# Autodesk Inventor assembly: Final assembly cuz we cool
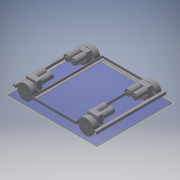
[picture p0: Inventor's stored thumbnail of the model, 180x180]
Saved by Autodesk Inventor 2016 SP2 (Build 200236200, 236)
## iProperties
Created: 2018-01-20
Part Number: Final assembly cuz we cool
Document SubType Name: Assembly
Designer: CAD
Author: CAD
## Documents named in this file (6)
- C:\Users\CAD\Documents\GitHub\FIRST-ROBOTICS-2018-5436-CAD\Robot\Chassis\Final assembly cuz we cool.iam
- C:\Users\CAD\Documents\GitHub\FIRST-ROBOTICS-2018-5436-CAD\Robot\Chassis\27.5 L.ipt
- C:\Users\CAD\Documents\GitHub\FIRST-ROBOTICS-2018-5436-CAD\Robot\Chassis\17.25 L.ipt
- C:\Users\CAD\Documents\GitHub\FIRST-ROBOTICS-2018-5436-CAD\Robot\Chassis\transmission with brackets.iam
- C:\Users\CAD\Documents\GitHub\FIRST-ROBOTICS-2018-5436-CAD\Robot\Chassis\Temp Wheels.ipt
- C:\Users\CAD\Documents\GitHub\FIRST-ROBOTICS-2018-5436-CAD\Robot\Chassis\27 in sq frame.ipt
## Components (14 placed, 5 different names)
1. 27.5 L:1 — Mate:9, Mate:10, Mate:25, Mate:26, Mate:29, Mate:30, Flush:2, Flush:3, Mate:32, Flush:4, Flush:5
2. transmission with brackets:1 [sub-assembly] — Mate:11, Mate:18, Mate:19, Mate:23
3. transmission with brackets:2 [sub-assembly] — Mate:10, Mate:12, Mate:17, Mate:20, Mate:24
4. transmission with brackets:3 [sub-assembly] — Mate:14, Mate:15, Mate:21
5. transmission with brackets:4 [sub-assembly] — Mate:9, Mate:13, Mate:16, Mate:22
6. Temp Wheels:1 — Mate:11, Mate:18, Mate:19
7. Temp Wheels:2 — Mate:13, Mate:16, Mate:22, Tangent:2
8. Temp Wheels:3 — Mate:14, Mate:15, Mate:21
9. Temp Wheels:4 — Mate:12, Mate:17, Mate:20
10. 27 in sq frame:1 — Mate:24
11. 27 in sq frame:2 — Mate:23, Angle:2
12. 17.25 L:1 — Mate:29, Mate:30, Flush:2, Mate:31, Flush:5, Mate:33, Flush:6
13. 17.25 L:2 — Mate:25, Mate:26, Flush:3, Mate:32, Flush:4
14. 27.5 L:2 — Mate:31, Mate:33, Flush:6
## Relationships (30: Mate 23, Flush 5, Angle 1, Tangent 1)
- Mate:9: 27.5 L:1 ↔ transmission with brackets:4
- Mate:10: 27.5 L:1 ↔ transmission with brackets:2
- Mate:11: transmission with brackets:1 ↔ Temp Wheels:1
- Mate:12: transmission with brackets:2 ↔ Temp Wheels:4
- Mate:13: transmission with brackets:4 ↔ Temp Wheels:2
- Mate:14: transmission with brackets:3 ↔ Temp Wheels:3
- Mate:15: transmission with brackets:3 ↔ Temp Wheels:3
- Mate:16: transmission with brackets:4 ↔ Temp Wheels:2
- Mate:17: transmission with brackets:2 ↔ Temp Wheels:4
- Mate:18: transmission with brackets:1 ↔ Temp Wheels:1
- Mate:19 (9.525 mm): transmission with brackets:1 ↔ Temp Wheels:1
- Mate:20 (9.525 mm): transmission with brackets:2 ↔ Temp Wheels:4
- Mate:21 (9.525 mm): transmission with brackets:3 ↔ Temp Wheels:3
- Mate:22 (9.525 mm): transmission with brackets:4 ↔ Temp Wheels:2
- Mate:23: transmission with brackets:1 ↔ 27 in sq frame:2
- Mate:24: transmission with brackets:2 ↔ 27 in sq frame:1
- Mate:25: 27.5 L:1 ↔ 17.25 L:2
- Mate:26: 27.5 L:1 ↔ 17.25 L:2
- Mate:29: 27.5 L:1 ↔ 17.25 L:1
- Mate:30: 27.5 L:1 ↔ 17.25 L:1
- Flush:2: 27.5 L:1 ↔ 17.25 L:1
- Flush:3: 27.5 L:1 ↔ 17.25 L:2
- Mate:31: 17.25 L:1 ↔ 27.5 L:2
- Mate:32: 27.5 L:1 ↔ 17.25 L:2
- Flush:4: 27.5 L:1 ↔ 17.25 L:2
- Flush:5: 27.5 L:1 ↔ 17.25 L:1
- Angle:2 (0 deg): 27 in sq frame:2
- Tangent:2: Temp Wheels:2
- Mate:33: 17.25 L:1 ↔ 27.5 L:2
- Flush:6: 17.25 L:1 ↔ 27.5 L:2
